# Autodesk Inventor assembly: Assembly1
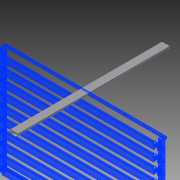
[picture p0: Inventor's stored thumbnail of the model, 180x180]
Saved by Autodesk Inventor 2015 SP1 (Build 190203100, 203)
## iProperties
Created: 2015-03-28
Part Number: Assembly1
Document SubType Name: Assembly
Designer: Cyril
Mass: 815.005 g
Surface Area: 4323.83 cm^2
Volume: 815.005 cm^3
Density: 1 g/cm^3
Author: Cyril
## Documents named in this file (11)
- C:\Users\Cyril\Documents\OSE FR\Concentrateur solaire\Inventor\Assemblage_miroir.iam
- C:\Users\Cyril\Documents\OSE FR\Concentrateur solaire\Inventor\Miroir.ipt
- C:\Users\Cyril\Documents\OSE FR\Concentrateur solaire\Inventor\Part3.ipt
- C:\Users\Cyril\Documents\OSE FR\Concentrateur solaire\Inventor\Tube sous miroir.ipt
- C:\Users\Cyril\Documents\OSE FR\Concentrateur solaire\Inventor\tige.ipt
- C:\Users\Cyril\Documents\OSE FR\Concentrateur solaire\Inventor\ecrou_nf_en_iso_4032_m4_6.ipt
- C:\Users\Cyril\Documents\OSE FR\Concentrateur solaire\Inventor\ecrou_nf_en_iso_4032_m4_6_MIR1.ipt
- C:\Users\Cyril\Documents\OSE FR\Concentrateur solaire\Inventor\Part3_MIR1.ipt
- C:\Users\Cyril\Documents\OSE FR\Concentrateur solaire\Inventor\tige_MIR1.ipt
- C:\Users\Cyril\Documents\OSE FR\Concentrateur solaire\Inventor\ecrou_nf_en_iso_4032_m4_6_MIR2.ipt
- C:\Users\Cyril\Documents\OSE FR\Concentrateur solaire\Inventor\ecrou_nf_en_iso_4032_m4_6_MIR1_MIR.ipt
## Components (10 placed, 10 different names)
1. Miroir:1 — Flush:4, Mate:13, Mate:14, Angle:1, Flush:7, Flush:8, Flush:9
2. Part3:1 — Mate:17, Flush:5, Flush:6, Angle:1
3. Tube sous miroir:1 — Flush:4, Mate:13, Mate:14, Mate:15, Mate:16, Flush:5
4. tige:1 — Mate:15, Mate:16, Mate:17, Mate:18
5. ecrou_nf_en_iso_4032_m4_6:1 — Mate:18, Flush:6
6. ecrou_nf_en_iso_4032_m4_6_MIR1:1
7. Part3_MIR1:1 — Mate:19, Flush:10
8. tige_MIR1:1 — Mate:19, Mate:20
9. ecrou_nf_en_iso_4032_m4_6_MIR2:1 — Flush:10, Mate:20
10. ecrou_nf_en_iso_4032_m4_6_MIR1_MIR:1
## Relationships (16: Mate 8, Flush 7, Angle 1)
- Flush:4: Miroir:1 ↔ Tube sous miroir:1
- Mate:13: Miroir:1 ↔ Tube sous miroir:1
- Mate:14: Miroir:1 ↔ Tube sous miroir:1
- Mate:15: Tube sous miroir:1 ↔ tige:1
- Mate:16: Tube sous miroir:1 ↔ tige:1
- Mate:17: Part3:1 ↔ tige:1
- Flush:5: Part3:1 ↔ Tube sous miroir:1
- Mate:18: tige:1 ↔ ecrou_nf_en_iso_4032_m4_6:1
- Flush:6 (47.2 mm): Part3:1 ↔ ecrou_nf_en_iso_4032_m4_6:1
- Angle:1 (0 deg): Miroir:1 ↔ Part3:1
- Flush:7: Miroir:1
- Flush:8: Miroir:1
- Flush:9: Miroir:1
- Mate:19: Part3_MIR1:1 ↔ tige_MIR1:1
- Flush:10 (47.2 mm): Part3_MIR1:1 ↔ ecrou_nf_en_iso_4032_m4_6_MIR2:1
- Mate:20: tige_MIR1:1 ↔ ecrou_nf_en_iso_4032_m4_6_MIR2:1
